# Autodesk Inventor assembly: NanoAndPlate
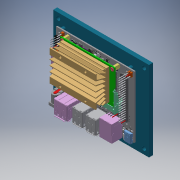
[picture p0: Inventor's stored thumbnail of the model, 180x180]
Saved by Autodesk Inventor 2019 (Build 230136000, 136)
## iProperties
Created: 2019-12-14
Part Number: NanoAndPlate
Document SubType Name: Assembly
Designer: james
Author: james
## Documents named in this file (3)
- F:\JimsRobot\FIRSTRobots\Design\Library\Jims\NanoAndPlate.iam
- F:\JimsRobot\FIRSTRobots\Design\Library\Jims\JetsonPlate.ipt
- F:\JimsRobot\FIRSTRobots\Design\Library\NVIDIA\Nano\P3450_P3449_A02_P3448_A02.iam
## Components (2 placed, 2 different names)
1. JetsonPlate:1 — Mate:1, Mate:2, Mate:3
2. P3450_P3449_A02_P3448_A02:1 [sub-assembly] — Mate:1, Mate:2, Mate:3
## Relationships (3: Mate 3)
- Mate:1: JetsonPlate:1 ↔ P3450_P3449_A02_P3448_A02:1
- Mate:2: JetsonPlate:1 ↔ P3450_P3449_A02_P3448_A02:1
- Mate:3: JetsonPlate:1 ↔ P3450_P3449_A02_P3448_A02:1
